# Autodesk Inventor assembly: noga_pre_MIR
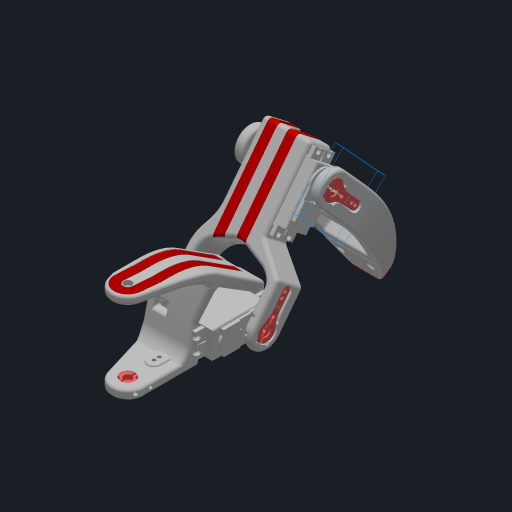
[picture p0: Inventor's stored thumbnail of the model, 512x512]
Saved by Autodesk Inventor 2023.4 (Build 274418000, 418)
## iProperties
Created: 2024-06-27
Part Number: noga_pre_MIR
Document SubType Name: Assembly
Designer: komputer
Author: kamil
## Documents named in this file (11)
- E:\PROJECTS_REPOS\Robal-2.0\mechanics\noga_pre_MIR.iam
- E:\PROJECTS_REPOS\Robal-2.0\mechanics\Standard-Servo_MIR.ipt
- E:\PROJECTS_REPOS\Robal-2.0\mechanics\czlon2_pre_MIR.ipt
- E:\PROJECTS_REPOS\Robal-2.0\mechanics\czlon3_pre_MIR.ipt
- E:\PROJECTS_REPOS\Robal-2.0\mechanics\SERVO ARM HORN 25T ALUMINIUM\SERVO ARM HORN 25T ALUMINIUM_MIR.ipt
- E:\PROJECTS_REPOS\Robal-2.0\mechanics\czlon_2_wciecie_1_MIR.ipt
- E:\PROJECTS_REPOS\Robal-2.0\mechanics\czlon_2_wciecie_2_MIR.ipt
- E:\PROJECTS_REPOS\Robal-2.0\mechanics\czlon_2_wciecie_3_MIR.ipt
- E:\PROJECTS_REPOS\Robal-2.0\mechanics\czlon_3_wciecie_1_MIR.ipt
- E:\PROJECTS_REPOS\Robal-2.0\mechanics\czlon_3_wciecie_2_MIR.ipt
- E:\PROJECTS_REPOS\Robal-2.0\mechanics\czlon_4_zloz_MIR.iam
## Components (13 placed, 10 different names)
1. Standard-Servo_MIR:1 — Mate:26, Mate:11, Mate:9, Mate:25, Mate:24
2. czlon2_pre_MIR:1 — Mate:26, Mate:11, Mate:9, Mate:49, Mate:48, Angle:1, Mate:37, Mate:33, Mate:32, Mate:36, Mate:35, Mate:39, Mate:38
3. czlon3_pre_MIR:1 — Mate:49, Mate:48, Mate:59, Mate:58, Angle:6, Mate:52, Mate:51, Mate:50, Mate:56, Mate:55, Mate:53, Mate:57, Mate:54
4. Standard-Servo_MIR:2 — Mate:59, Mate:58, Mate:46, Mate:47
5. SERVO ARM HORN 25T ALUMINIUM_MIR:1 — Angle:1
6. SERVO ARM HORN 25T ALUMINIUM_MIR:2 — Angle:6, Mate:25, Mate:24, Flush:5
7. czlon_2_wciecie_1_MIR:1 — Mate:37, Mate:33, Mate:32, Angle:3
8. czlon_2_wciecie_2_MIR:1 — Mate:36, Mate:35
9. czlon_2_wciecie_3_MIR:1 — Angle:3, Mate:39, Mate:38
10. czlon_3_wciecie_1_MIR:1 — Mate:52, Mate:51, Mate:50
11. czlon_3_wciecie_2_MIR:1 — Mate:56, Mate:55, Mate:53
12. SERVO ARM HORN 25T ALUMINIUM_MIR:3 — Mate:46, Flush:5
13. czlon_4_zloz_MIR:1 [sub-assembly] — Mate:57, Mate:54, Mate:47
## Relationships (30: Mate 26, Angle 3, Flush 1)
- Mate:26: Standard-Servo_MIR:1 ↔ czlon2_pre_MIR:1
- Mate:11: Standard-Servo_MIR:1 ↔ czlon2_pre_MIR:1
- Mate:9 (1 mm): Standard-Servo_MIR:1 ↔ czlon2_pre_MIR:1
- Mate:49: czlon2_pre_MIR:1 ↔ czlon3_pre_MIR:1
- Mate:48 (2 mm): czlon2_pre_MIR:1 ↔ czlon3_pre_MIR:1
- Mate:59: czlon3_pre_MIR:1 ↔ Standard-Servo_MIR:2
- Mate:58: czlon3_pre_MIR:1 ↔ Standard-Servo_MIR:2
- Angle:1 (0 deg): czlon2_pre_MIR:1 ↔ SERVO ARM HORN 25T ALUMINIUM_MIR:1
- Angle:6 (180 deg): czlon3_pre_MIR:1 ↔ SERVO ARM HORN 25T ALUMINIUM_MIR:2
- Mate:25: Standard-Servo_MIR:1 ↔ SERVO ARM HORN 25T ALUMINIUM_MIR:2
- Mate:24: Standard-Servo_MIR:1 ↔ SERVO ARM HORN 25T ALUMINIUM_MIR:2
- Mate:37 (0.1 mm): czlon2_pre_MIR:1 ↔ czlon_2_wciecie_1_MIR:1
- Mate:33: czlon2_pre_MIR:1 ↔ czlon_2_wciecie_1_MIR:1
- Mate:32: czlon2_pre_MIR:1 ↔ czlon_2_wciecie_1_MIR:1
- Mate:36: czlon2_pre_MIR:1 ↔ czlon_2_wciecie_2_MIR:1
- Mate:35: czlon2_pre_MIR:1 ↔ czlon_2_wciecie_2_MIR:1
- Angle:3 (180 deg): czlon_2_wciecie_1_MIR:1 ↔ czlon_2_wciecie_3_MIR:1
- Mate:39: czlon2_pre_MIR:1 ↔ czlon_2_wciecie_3_MIR:1
- Mate:38: czlon2_pre_MIR:1 ↔ czlon_2_wciecie_3_MIR:1
- Mate:52: czlon3_pre_MIR:1 ↔ czlon_3_wciecie_1_MIR:1
- Mate:51: czlon3_pre_MIR:1 ↔ czlon_3_wciecie_1_MIR:1
- Mate:50: czlon3_pre_MIR:1 ↔ czlon_3_wciecie_1_MIR:1
- Mate:56: czlon3_pre_MIR:1 ↔ czlon_3_wciecie_2_MIR:1
- Mate:55: czlon3_pre_MIR:1 ↔ czlon_3_wciecie_2_MIR:1
- Mate:53: czlon3_pre_MIR:1 ↔ czlon_3_wciecie_2_MIR:1
- Mate:46: Standard-Servo_MIR:2 ↔ SERVO ARM HORN 25T ALUMINIUM_MIR:3
- Flush:5: SERVO ARM HORN 25T ALUMINIUM_MIR:2 ↔ SERVO ARM HORN 25T ALUMINIUM_MIR:3
- Mate:57 (2 mm): czlon3_pre_MIR:1 ↔ czlon_4_zloz_MIR:1
- Mate:54: czlon3_pre_MIR:1 ↔ czlon_4_zloz_MIR:1
- Mate:47 (0.1 mm): Standard-Servo_MIR:2 ↔ czlon_4_zloz_MIR:1
